# Autodesk Inventor assembly: Electrical Board 2
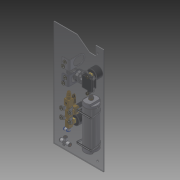
[picture p0: Inventor's stored thumbnail of the model, 180x180]
Saved by Autodesk Inventor 2014 SP1 (Build 180222100, 222)
## iProperties
Created: 2013-12-13
Part Number: Electrical Board 2
Document SubType Name: Assembly
Designer: Moses
Mass: 1240.84 g
Surface Area: 3277.63 cm^2
Volume: 609.67 cm^3
Density: 2.03527 g/cm^3
Author: Moses
## Documents named in this file (23)
- C:\Users\Moses\Documents\Inventor\Sally Rebuild\Rebuild Sally\Electrical Board 2.iam
- C:\Users\Moses\Documents\Inventor\Sally Rebuild\Rebuild Sally\Electrical Board 2.ipt
- C:\Users\Moses\Documents\Inventor\Sally Rebuild\Rebuild Sally\CS_Relay_SPIKE-RELAY-H.ipt
- C:\Users\Moses\Documents\Inventor\Sally Rebuild\Rebuild Sally\Pneumatics\Pneumatics_SMC_KQ2T07-00.ipt
- C:\Users\Moses\Documents\Inventor\Sally Rebuild\Rebuild Sally\Pneumatics\Pneumatics_Parker_PV609-2.ipt
- C:\Users\Moses\Documents\Inventor\Sally Rebuild\Rebuild Sally\Pneumatics\Pneumatics_Clippard_AVT-32-16.iam
- C:\Users\Moses\Documents\Inventor\Sally Rebuild\Rebuild Sally\Pneumatics\Pneumatics_Norgren_R07-100-RNEA.ipt
- C:\Users\Moses\Documents\Inventor\Sally Rebuild\Rebuild Sally\Pneumatics\Pneumatics_Monnier_13536_Mounting Bracket.ipt
- C:\Users\Moses\Documents\Inventor\Sally Rebuild\Rebuild Sally\Pneumatics\Pneumatics_SMC_KQ2H03-34S.ipt
- C:\Users\Moses\Documents\Inventor\Sally Rebuild\Rebuild Sally\Pneumatics\Pneumatics_NASON_SM-2B-115R.ipt
- C:\Users\Moses\Documents\Inventor\Sally Rebuild\Rebuild Sally\Pneumatics\Pneumatics_Parker_2203P-2.ipt
- C:\Users\Moses\Documents\Inventor\Sally Rebuild\Rebuild Sally\Pneumatics\Pneumatics_Parker_216P-2.ipt
- C:\Users\Moses\Documents\Inventor\Sally Rebuild\Rebuild Sally\Pneumatics\Pneumatics_SMC_KQ2L03-34S.ipt
- C:\Users\Moses\Documents\Inventor\Sally Rebuild\Rebuild Sally\Pneumatics\Pneumatics_WIKA_9690242.ipt
- C:\Users\Moses\Documents\Inventor\Sally Rebuild\Rebuild Sally\Pneumatics\Pneumatics_SMC_KQ2H07-35S.ipt
- C:\Users\Moses\Documents\Inventor\Sally Rebuild\Rebuild Sally\Clippard Zip Tie 2.ipt
- C:\Users\Moses\Documents\Inventor\Sally Rebuild\Rebuild Sally\Standard #10 Washer.ipt
- C:\Users\Moses\Documents\Inventor\Sally Rebuild\Rebuild Sally\Pneumatics\Pneumatics_Norgren_18-025-003_Bracket.ipt
- C:\Users\Moses\Documents\Inventor\Sally Rebuild\Rebuild Sally\Pneumatics\Pneumatics_Norgren_18-025-003_Panel Nut.ipt
- C:\Users\Moses\Documents\Inventor\Sally Rebuild\Rebuild Sally\Pneumatics Steel Bracket.ipt
- C:\Users\Moses\Documents\Inventor\Sally Rebuild\Rebuild Sally\90715A007.ipt
- C:\Users\Moses\Documents\Inventor\Sally Rebuild\Rebuild Sally\Standard #6 Washer.ipt
- C:\Users\Moses\Documents\Inventor\Sally Rebuild\Rebuild Sally\6-32 18-8 Stainless Steel Pan Head Philips Machine Screw\0.6250\91772A150.ipt
## Components (40 placed, 22 different names)
1. Electrical Board 2:1 — Mate:1, Tangent:1, Mate:2, Mate:3, Mate:4, Mate:5, Mate:6, Mate:7, Mate:8, Angle:1, Mate:11, Mate:12, Mate:13, Mate:14, Angle:3, Angle:5, Angle:7, Angle:8, Tangent:2, Tangent:3, Tangent:4, Tangent:5, Flush:2, Insert:12, Insert:13, Insert:14, Insert:15, Mate:21, Mate:22, Mate:25, Mate:26, Insert:16, Insert:17, Insert:18, Insert:19, Insert:22, Insert:23
2. CS_Relay_SPIKE-RELAY-H:1 — Mate:1, Mate:2, Mate:3, Insert:24, Insert:25
3. Pneumatics_SMC_KQ2T07-00:1 — Mate:7, Mate:8, Angle:1
4. Pneumatics_Parker_PV609-2:1 — Mate:14, Insert:1, Insert:3, Angle:2, Angle:3
5. Pneumatics_Clippard_AVT-32-16:1 [sub-assembly] — Tangent:1, Insert:10, Insert:11, Mate:16, Mate:17, Flush:2
6. Pneumatics_Norgren_18-025-003_Bracket:1 — Mate:4, Mate:5, Mate:6, Mate:9, Mate:10, Flush:3, Mate:18, Mate:20
7. Pneumatics_Norgren_R07-100-RNEA:1 — Mate:9, Mate:10, Insert:9, Mate:19
8. Pneumatics_Monnier_13536_Mounting Bracket:2 — Mate:11, Mate:12, Mate:13, Flush:3, Mate:18
9. Pneumatics_SMC_KQ2H03-34S:1 — Insert:1
10. Pneumatics_NASON_SM-2B-115R:1 — Insert:4
11. Pneumatics_Parker_2203P-2:1 — Insert:2, Insert:4, Angle:2, Insert:5, Angle:4, Tangent:6, Mate:23, Mate:24
12. Pneumatics_Parker_216P-2:1 — Insert:2, Insert:3
13. Pneumatics_Parker_216P-2:2 — Insert:5, Insert:6
14. Pneumatics_Parker_2203P-2:2 — Insert:6, Angle:4, Insert:7, Insert:8, Angle:6
15. Pneumatics_SMC_KQ2L03-34S:1 — Insert:7, Angle:5
16. Pneumatics_WIKA_9690242:1 — Insert:8, Angle:6
17. Pneumatics_WIKA_9690242:2 — Insert:9
18. Pneumatics_SMC_KQ2H07-35S:1 — Insert:10
19. Pneumatics_SMC_KQ2H07-35S:2 — Insert:11
20. Clippard Zip Tie 2:1 — Mate:16, Angle:7, Tangent:2, Tangent:4
21. Clippard Zip Tie 2:2 — Mate:17, Angle:8, Tangent:3, Tangent:5
22. Standard #10 Washer:1 — Insert:12
23. Standard #10 Washer:2 — Insert:13
24. Standard #10 Washer:3 — Insert:14
25. Standard #10 Washer:4 — Insert:15
26. Pneumatics_Norgren_18-025-003_Panel Nut:1 — Mate:19, Mate:20
27. Pneumatics Steel Bracket:1 — Mate:21, Flush:4, Mate:23, Mate:26
28. Pneumatics Steel Bracket:2 — Mate:22, Tangent:6, Flush:4, Mate:24, Mate:25
29. Standard #10 Washer:5 — Insert:16
30. Standard #10 Washer:6 — Insert:19
31. Standard #10 Washer:7 — Insert:18
32. Standard #10 Washer:8 — Insert:17
33. 90715A007:1 — Insert:21
34. 90715A007:2 — Insert:20
35. Standard #6 Washer:1 — Insert:21, Insert:22
36. Standard #6 Washer:2 — Insert:20, Insert:23
37. Standard #6 Washer:3 — Insert:24, Insert:26
38. Standard #6 Washer:4 — Insert:25, Insert:27
39. 91772A150:1 — Insert:26
40. 91772A150:2 — Insert:27
## Relationships (69: Insert 27, Mate 25, Angle 8, Tangent 6, Flush 3)
- Mate:1: Electrical Board 2:1 ↔ CS_Relay_SPIKE-RELAY-H:1
- Tangent:1: Electrical Board 2:1 ↔ Pneumatics_Clippard_AVT-32-16:1
- Mate:2: Electrical Board 2:1 ↔ CS_Relay_SPIKE-RELAY-H:1
- Mate:3: Electrical Board 2:1 ↔ CS_Relay_SPIKE-RELAY-H:1
- Mate:4: Electrical Board 2:1 ↔ Pneumatics_Norgren_18-025-003_Bracket:1
- Mate:5: Electrical Board 2:1 ↔ Pneumatics_Norgren_18-025-003_Bracket:1
- Mate:6: Electrical Board 2:1 ↔ Pneumatics_Norgren_18-025-003_Bracket:1
- Mate:7: Electrical Board 2:1 ↔ Pneumatics_SMC_KQ2T07-00:1
- Mate:8: Electrical Board 2:1 ↔ Pneumatics_SMC_KQ2T07-00:1
- Angle:1 (0 deg): Electrical Board 2:1 ↔ Pneumatics_SMC_KQ2T07-00:1
- Mate:9: Pneumatics_Norgren_18-025-003_Bracket:1 ↔ Pneumatics_Norgren_R07-100-RNEA:1
- Mate:10: Pneumatics_Norgren_18-025-003_Bracket:1 ↔ Pneumatics_Norgren_R07-100-RNEA:1
- Mate:11: Electrical Board 2:1 ↔ Pneumatics_Monnier_13536_Mounting Bracket:2
- Mate:12: Electrical Board 2:1 ↔ Pneumatics_Monnier_13536_Mounting Bracket:2
- Mate:13: Electrical Board 2:1 ↔ Pneumatics_Monnier_13536_Mounting Bracket:2
- Mate:14: Electrical Board 2:1 ↔ Pneumatics_Parker_PV609-2:1
- Insert:1 (1.27 mm): Pneumatics_Parker_PV609-2:1 ↔ Pneumatics_SMC_KQ2H03-34S:1
- Insert:2 (1.27 mm): Pneumatics_Parker_2203P-2:1 ↔ Pneumatics_Parker_216P-2:1
- Insert:3 (1.27 mm): Pneumatics_Parker_PV609-2:1 ↔ Pneumatics_Parker_216P-2:1
- Insert:4 (-1.27 mm): Pneumatics_NASON_SM-2B-115R:1 ↔ Pneumatics_Parker_2203P-2:1
- Angle:2 (0 deg): Pneumatics_Parker_PV609-2:1 ↔ Pneumatics_Parker_2203P-2:1
- Angle:3 (0 deg): Electrical Board 2:1 ↔ Pneumatics_Parker_PV609-2:1
- Insert:5 (2.54 mm): Pneumatics_Parker_2203P-2:1 ↔ Pneumatics_Parker_216P-2:2
- Insert:6 (2.54 mm): Pneumatics_Parker_216P-2:2 ↔ Pneumatics_Parker_2203P-2:2
- Angle:4 (0 deg): Pneumatics_Parker_2203P-2:1 ↔ Pneumatics_Parker_2203P-2:2
- Insert:7 (1.27 mm): Pneumatics_Parker_2203P-2:2 ↔ Pneumatics_SMC_KQ2L03-34S:1
- Angle:5 (0 deg): Electrical Board 2:1 ↔ Pneumatics_SMC_KQ2L03-34S:1
- Insert:8 (1.27 mm): Pneumatics_Parker_2203P-2:2 ↔ Pneumatics_WIKA_9690242:1
- Angle:6 (0 deg): Pneumatics_Parker_2203P-2:2 ↔ Pneumatics_WIKA_9690242:1
- Insert:9 (1.27 mm): Pneumatics_Norgren_R07-100-RNEA:1 ↔ Pneumatics_WIKA_9690242:2
- Insert:10 (1.27 mm): Pneumatics_Clippard_AVT-32-16:1 ↔ Pneumatics_SMC_KQ2H07-35S:1
- Insert:11 (1.27 mm): Pneumatics_Clippard_AVT-32-16:1 ↔ Pneumatics_SMC_KQ2H07-35S:2
- Mate:16: Pneumatics_Clippard_AVT-32-16:1 ↔ Clippard Zip Tie 2:1
- Angle:7 (0 deg): Electrical Board 2:1 ↔ Clippard Zip Tie 2:1
- Mate:17: Pneumatics_Clippard_AVT-32-16:1 ↔ Clippard Zip Tie 2:2
- Angle:8 (0 deg): Electrical Board 2:1 ↔ Clippard Zip Tie 2:2
- Tangent:2 (-5.334 mm): Electrical Board 2:1 ↔ Clippard Zip Tie 2:1
- Tangent:3 (-5.334 mm): Electrical Board 2:1 ↔ Clippard Zip Tie 2:2
- Tangent:4 (-0.635 mm): Electrical Board 2:1 ↔ Clippard Zip Tie 2:1
- Tangent:5 (-0.635 mm): Electrical Board 2:1 ↔ Clippard Zip Tie 2:2
- Flush:2 (25.4 mm): Electrical Board 2:1 ↔ Pneumatics_Clippard_AVT-32-16:1
- Insert:12: Electrical Board 2:1 ↔ Standard #10 Washer:1
- Insert:13: Electrical Board 2:1 ↔ Standard #10 Washer:2
- Insert:14: Electrical Board 2:1 ↔ Standard #10 Washer:3
- Insert:15: Electrical Board 2:1 ↔ Standard #10 Washer:4
- Flush:3: Pneumatics_Norgren_18-025-003_Bracket:1 ↔ Pneumatics_Monnier_13536_Mounting Bracket:2
- Mate:18 (19.05 mm): Pneumatics_Norgren_18-025-003_Bracket:1 ↔ Pneumatics_Monnier_13536_Mounting Bracket:2
- Mate:19: Pneumatics_Norgren_R07-100-RNEA:1 ↔ Pneumatics_Norgren_18-025-003_Panel Nut:1
- Mate:20: Pneumatics_Norgren_18-025-003_Bracket:1 ↔ Pneumatics_Norgren_18-025-003_Panel Nut:1
- Mate:21: Electrical Board 2:1 ↔ Pneumatics Steel Bracket:1
- Mate:22: Electrical Board 2:1 ↔ Pneumatics Steel Bracket:2
- Tangent:6: Pneumatics_Parker_2203P-2:1 ↔ Pneumatics Steel Bracket:2
- Flush:4: Pneumatics Steel Bracket:1 ↔ Pneumatics Steel Bracket:2
- Mate:23 (3.175 mm): Pneumatics_Parker_2203P-2:1 ↔ Pneumatics Steel Bracket:1
- Mate:24 (3.175 mm): Pneumatics_Parker_2203P-2:1 ↔ Pneumatics Steel Bracket:2
- Mate:25: Electrical Board 2:1 ↔ Pneumatics Steel Bracket:2
- Mate:26: Electrical Board 2:1 ↔ Pneumatics Steel Bracket:1
- Insert:16: Electrical Board 2:1 ↔ Standard #10 Washer:5
- Insert:17: Electrical Board 2:1 ↔ Standard #10 Washer:8
- Insert:18: Electrical Board 2:1 ↔ Standard #10 Washer:7
- Insert:19: Electrical Board 2:1 ↔ Standard #10 Washer:6
- Insert:20: 90715A007:2 ↔ Standard #6 Washer:2
- Insert:21: 90715A007:1 ↔ Standard #6 Washer:1
- Insert:22: Electrical Board 2:1 ↔ Standard #6 Washer:1
- Insert:23: Electrical Board 2:1 ↔ Standard #6 Washer:2
- Insert:24: CS_Relay_SPIKE-RELAY-H:1 ↔ Standard #6 Washer:3
- Insert:25: CS_Relay_SPIKE-RELAY-H:1 ↔ Standard #6 Washer:4
- Insert:26: Standard #6 Washer:3 ↔ 91772A150:1
- Insert:27: Standard #6 Washer:4 ↔ 91772A150:2
